# Autodesk Inventor assembly: Upper_Leg_Right
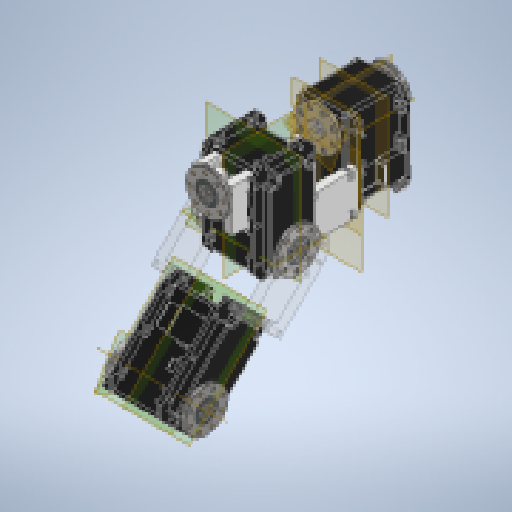
[picture p0: Inventor's stored thumbnail of the model, 512x512]
Saved by Autodesk Inventor 2024 (Build 280153000, 153)
## iProperties
Created: 2024-09-17
Part Number: Upper_Leg_Right
Document SubType Name: Assembly
Designer: Eungang
Author: Eungang
## Documents named in this file (8)
- C:\Users\Eungang\Documents\Inventor\FIGHTING_ROBOT_FINAL\부품\Upper_Leg_Right\Upper_Leg_Right.iam
- C:\Users\Eungang\Documents\Inventor\FIGHTING_ROBOT_FINAL\64-106_connect.ipt
- C:\Users\Eungang\Documents\Inventor\FIGHTING_ROBOT_FINAL\부품\Upper_Leg_Right\MX-106T.ipt
- C:\Users\Eungang\Documents\Inventor\FIGHTING_ROBOT_FINAL\부품\아이들러\64아이들러.iam
- C:\Users\Eungang\Documents\Inventor\FIGHTING_ROBOT_FINAL\부품\혼\64-106Horn.ipt
- C:\Users\Eungang\Documents\Inventor\FIGHTING_ROBOT_FINAL\부품\Upper_Leg_Right\waist_thighs_bridge.ipt
- C:\Users\Eungang\Documents\Inventor\FIGHTING_ROBOT_FINAL\부품\다이나믹셀\MX-64T.ipt
- C:\Users\Eungang\Documents\Inventor\FIGHTING_ROBOT_FINAL\부품\Upper_Leg_Right\knee_thighs_connect.ipt
## Components (15 placed, 7 different names)
1. MX-106T:1 — 삽입:2, 삽입:4, 삽입:33, 삽입:34, 삽입:36, 삽입:37
2. 64아이들러:1 [sub-assembly] — 삽입:10, 삽입:32
3. 64-106Horn:1 — 삽입:11, 삽입:35, 삽입:38
4. 64아이들러:2 [sub-assembly] — 삽입:4
5. 64-106Horn:2 — 삽입:2
6. MX-106T:2 — 삽입:10, 삽입:11, 삽입:17, 삽입:18, 삽입:24, 삽입:25, 삽입:28, 삽입:29
7. waist_thighs_bridge:1 — 삽입:17, 삽입:18, 삽입:19
8. 64아이들러:3 [sub-assembly] — 삽입:19
9. MX-64T:1 — 삽입:22, 삽입:23, 삽입:26, 삽입:27
10. 64-106Horn:3 — 삽입:22
11. 64아이들러:4 [sub-assembly] — 삽입:23
12. 64-106_connect:1 — 삽입:24, 삽입:25, 삽입:26, 삽입:27
13. 64-106_connect:2 — 삽입:28, 삽입:29, 각도:1
14. knee_thighs_connect:1 — 삽입:32, 삽입:33, 삽입:34
15. knee_thighs_connect:2 — 삽입:35, 삽입:36, 삽입:37, 삽입:38, 각도:1
## Relationships (23: Insert 22, Angle 1)
- 삽입:2 [Insert] (0.5 mm): MX-106T:1 ↔ 64-106Horn:2
- 삽입:4 [Insert] (0.5 mm): MX-106T:1 ↔ 64아이들러:2
- 삽입:10 [Insert] (0.5 mm): 64아이들러:1 ↔ MX-106T:2
- 삽입:11 [Insert] (0.5 mm): 64-106Horn:1 ↔ MX-106T:2
- 삽입:17 [Insert] (0.1 mm): MX-106T:2 ↔ waist_thighs_bridge:1
- 삽입:18 [Insert] (0.1 mm): MX-106T:2 ↔ waist_thighs_bridge:1
- 삽입:19 [Insert]: waist_thighs_bridge:1 ↔ 64아이들러:3
- 삽입:22 [Insert] (0.5 mm): MX-64T:1 ↔ 64-106Horn:3
- 삽입:23 [Insert] (0.5 mm): MX-64T:1 ↔ 64아이들러:4
- 삽입:24 [Insert] (0.1 mm): MX-106T:2 ↔ 64-106_connect:1
- 삽입:25 [Insert] (0.1 mm): MX-106T:2 ↔ 64-106_connect:1
- 삽입:26 [Insert] (0.1 mm): MX-64T:1 ↔ 64-106_connect:1
- 삽입:27 [Insert] (0.1 mm): MX-64T:1 ↔ 64-106_connect:1
- 삽입:28 [Insert] (0.1 mm): MX-106T:2 ↔ 64-106_connect:2
- 삽입:29 [Insert] (0.1 mm): MX-106T:2 ↔ 64-106_connect:2
- 삽입:32 [Insert]: 64아이들러:1 ↔ knee_thighs_connect:1
- 삽입:33 [Insert] (0.2 mm): MX-106T:1 ↔ knee_thighs_connect:1
- 삽입:34 [Insert] (0.2 mm): MX-106T:1 ↔ knee_thighs_connect:1
- 삽입:35 [Insert]: 64-106Horn:1 ↔ knee_thighs_connect:2
- 삽입:36 [Insert] (0.2 mm): MX-106T:1 ↔ knee_thighs_connect:2
- 삽입:37 [Insert] (0.2 mm): MX-106T:1 ↔ knee_thighs_connect:2
- 삽입:38 [Insert]: 64-106Horn:1 ↔ knee_thighs_connect:2
- 각도:1 [Angle] (315 deg): 64-106_connect:2 ↔ knee_thighs_connect:2
